# Autodesk Inventor assembly: center cross-member
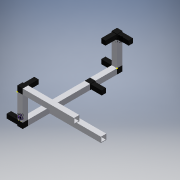
[picture p0: Inventor's stored thumbnail of the model, 180x180]
Saved by Autodesk Inventor 2017 (Build 210142000, 142)
## iProperties
Created: 2019-12-06
Part Number: center cross-member
Document SubType Name: Assembly
Designer: S346553810
Author: S346553810
## Documents named in this file (7)
- \\ad.ocdsb.ca\studenthome\3\S338674153\FRC 2020\FullRobotRefactor\SubFrame\center cross-member.iam
- \\ad.ocdsb.ca\studenthome\3\S338674153\FRC 2020\FullRobotRefactor\SubFrame\1in sq tub - 4.ipt
- \\ad.ocdsb.ca\studenthome\3\S338674153\FRC 2020\FullRobotRefactor\SubFrame\Kipp K0617.ipt
- \\ad.ocdsb.ca\studenthome\3\S338674153\FRC 2020\FullRobotRefactor\SubFrame\Kipp K0619.ipt
- \\ad.ocdsb.ca\studenthome\3\S338674153\FRC 2020\FullRobotRefactor\SubFrame\1in sq tub - 6.ipt
- \\ad.ocdsb.ca\studenthome\3\S338674153\FRC 2020\FullRobotRefactor\SubFrame\1in sq tub - 4-5.ipt
- \\ad.ocdsb.ca\studenthome\3\S338674153\FRC 2020\FullRobotRefactor\SubFrame\1in sq tub - 6-5.ipt
## Components (13 placed, 6 different names)
1. 1in sq tub - 4:1 — Mate:4, Flush:7, Flush:8
2. 1in sq tub - 4:2
3. Kipp K0617:1 — Mate:3, Flush:5, Flush:6, Mate:4, Flush:7, Flush:8
4. Kipp K0617:2
5. Kipp K0619:1
6. Kipp K0619:2
7. 1in sq tub - 6:2 — Mate:3, Flush:5, Flush:6
8. 1in sq tub - 4-5:1 — Mate:5, Flush:9, Flush:10
9. 1in sq tub - 4-5:2 — Flush:11, Mate:6, Flush:12
10. 1in sq tub - 6:3
11. 1in sq tub - 6-5:1
12. Kipp K0619:3 — Mate:5, Flush:9, Flush:10
13. Kipp K0619:4 — Flush:11, Mate:6, Flush:12
## Relationships (12: Flush 8, Mate 4)
- Mate:3: Kipp K0617:1 ↔ 1in sq tub - 6:2
- Flush:5: Kipp K0617:1 ↔ 1in sq tub - 6:2
- Flush:6: Kipp K0617:1 ↔ 1in sq tub - 6:2
- Mate:4: 1in sq tub - 4:1 ↔ Kipp K0617:1
- Flush:7: 1in sq tub - 4:1 ↔ Kipp K0617:1
- Flush:8: 1in sq tub - 4:1 ↔ Kipp K0617:1
- Mate:5: 1in sq tub - 4-5:1 ↔ Kipp K0619:3
- Flush:9: 1in sq tub - 4-5:1 ↔ Kipp K0619:3
- Flush:10: 1in sq tub - 4-5:1 ↔ Kipp K0619:3
- Flush:11: 1in sq tub - 4-5:2 ↔ Kipp K0619:4
- Mate:6: 1in sq tub - 4-5:2 ↔ Kipp K0619:4
- Flush:12: 1in sq tub - 4-5:2 ↔ Kipp K0619:4
